# Autodesk Inventor assembly: drive side + wheels
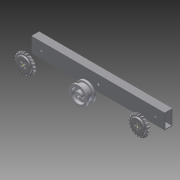
[picture p0: Inventor's stored thumbnail of the model, 180x180]
Saved by Autodesk Inventor 2015 (Build 190159000, 159)
## iProperties
Created: 2015-10-07
Part Number: drive side + wheels
Document SubType Name: Assembly
Designer: alhohbein
Author: alhohbein
## Documents named in this file (3)
- U:\drive side + wheels.iam
- U:\Drive base.ipt
- U:\Drive Train.iam
## Components (2 placed, 2 different names)
1. Drive base:1 — Mate:1, Mate:2
2. Drive Train:1 [sub-assembly] — Mate:1, Mate:2
## Relationships (2: Mate 2)
- Mate:1: Drive base:1 ↔ Drive Train:1
- Mate:2: Drive base:1 ↔ Drive Train:1
